# Autodesk Inventor assembly: Картер всборе
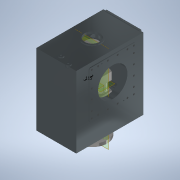
[picture p0: Inventor's stored thumbnail of the model, 180x180]
Saved by Autodesk Inventor 2021 (Build 250183000, 183)
## iProperties
Created: 2020-12-05
Part Number: Картер всборе
Document SubType Name: Assembly
Designer: Тимоха
Author: Тимоха
## Documents named in this file (12)
- C:\Users\Тимоха\Desktop\КР Компрессор\compressor\Картер всборе.iam
- C:\Users\Тимоха\Desktop\КР Компрессор\compressor\Картер.ipt
- C:\Users\Тимоха\Desktop\КР Компрессор\compressor\Крышка коренного подшипника1.ipt
- C:\Users\Тимоха\Desktop\КР Компрессор\compressor\Балка.ipt
- C:\Users\Тимоха\Desktop\КР Компрессор\compressor\Крышка стенки картера низ.ipt
- C:\Users\Тимоха\Desktop\КР Компрессор\compressor\Нижняя часть коренного подшипника.ipt
- C:\Users\Тимоха\Desktop\КР Компрессор\compressor\Вал.ipt
- C:\Users\Тимоха\Desktop\КР Компрессор\compressor\Крышка стенки картера верх.ipt
- C:\Users\Тимоха\Desktop\КР Компрессор\compressor\Крышка коренного подшипника.ipt
- C:\Users\Тимоха\Desktop\КР Компрессор\compressor\Крышка картера 1.ipt
- C:\Users\Тимоха\Desktop\КР Компрессор\compressor\Крышка картера 2.ipt
- C:\Users\Тимоха\Desktop\КР Компрессор\compressor\Крышка картера 3.ipt
## Components (15 placed, 11 different names)
1. Картер:1 — Заподлицо:3, Заподлицо:4, Жесткий:4, Жесткий:6, Совмещение:2, Заподлицо:7, Заподлицо:8, Жесткий:8, Заподлицо:9, Заподлицо:10, Заподлицо:11, Заподлицо:12, Заподлицо:13, Заподлицо:14
2. Балка:1
3. Балка:2
4. Крышка стенки картера низ:1 — Заподлицо:3, Заподлицо:4
5. Нижняя часть коренного подшипника:2 — Жесткий:4, Цилиндрический:1
6. Нижняя часть коренного подшипника:3 — Жесткий:6, Цилиндрический:2, Жесткий:7
7. Вал:1 — Цилиндрический:1, Цилиндрический:2, Совмещение:2
8. Нижняя часть коренного подшипника:4
9. Крышка стенки картера верх:1 — Заподлицо:7, Заподлицо:8
10. Крышка коренного подшипника:1
11. Крышка коренного подшипника1:2 — Жесткий:8
12. Нижняя часть коренного подшипника:5 — Жесткий:7
13. Крышка картера 1:1 — Заподлицо:9, Заподлицо:10
14. Крышка картера 2:1 — Заподлицо:11, Заподлицо:12
15. Крышка картера 3:1 — Заподлицо:13, Заподлицо:14
## Relationships (17: Flush 10, WeldJoint 4, CylindricalJoint 2, Mate 1)
- Заподлицо:3 [Flush]: Картер:1 ↔ Крышка стенки картера низ:1
- Заподлицо:4 [Flush]: Картер:1 ↔ Крышка стенки картера низ:1
- Жесткий:4 [WeldJoint]: Картер:1 ↔ Нижняя часть коренного подшипника:2
- Жесткий:6 [WeldJoint]: Картер:1 ↔ Нижняя часть коренного подшипника:3
- Цилиндрический:1 [CylindricalJoint]: Нижняя часть коренного подшипника:2 ↔ Вал:1
- Цилиндрический:2 [CylindricalJoint]: Нижняя часть коренного подшипника:3 ↔ Вал:1
- Совмещение:2 [Mate] (5 mm): Картер:1 ↔ Вал:1
- Заподлицо:7 [Flush]: Картер:1 ↔ Крышка стенки картера верх:1
- Заподлицо:8 [Flush]: Картер:1 ↔ Крышка стенки картера верх:1
- Жесткий:7 [WeldJoint]: Нижняя часть коренного подшипника:3 ↔ Нижняя часть коренного подшипника:5
- Жесткий:8 [WeldJoint]: Картер:1 ↔ Крышка коренного подшипника1:2
- Заподлицо:9 [Flush]: Картер:1 ↔ Крышка картера 1:1
- Заподлицо:10 [Flush]: Картер:1 ↔ Крышка картера 1:1
- Заподлицо:11 [Flush]: Картер:1 ↔ Крышка картера 2:1
- Заподлицо:12 [Flush]: Картер:1 ↔ Крышка картера 2:1
- Заподлицо:13 [Flush]: Картер:1 ↔ Крышка картера 3:1
- Заподлицо:14 [Flush]: Картер:1 ↔ Крышка картера 3:1
